# Autodesk Inventor assembly: my1020_motor
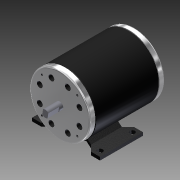
[picture p0: Inventor's stored thumbnail of the model, 180x180]
Saved by Autodesk Inventor 2012 (Build 160160000, 160)
## iProperties
Created: 2012-01-29
Part Number: my1020_motor
Document SubType Name: Assembly
Designer: Antonella Wilby
Author: Antonella Wilby
## Documents named in this file (4)
- E:\GCC Robotics 2012 - Mechanical\Robot 2.0\Drive Train\MY1020 Motor\my1020_motor.iam
- E:\GCC Robotics 2012 - Mechanical\Robot 2.0\Drive Train\MY1020 Motor\my1020_motor.ipt
- E:\GCC Robotics 2012 - Mechanical\Robot 2.0\Drive Train\MY1020 Motor\shaft.ipt
- E:\GCC Robotics 2012 - Mechanical\Robot 2.0\Drive Train\MY1020 Motor\mount plate.ipt
## Components (3 placed, 3 different names)
1. my1020_motor:1 — Mate:1, Mate:2, Mate:4, Mate:5, Flush:1
2. shaft:1 — Mate:1, Mate:2
3. mount plate:1 — Mate:4, Mate:5, Flush:1
## Relationships (5: Mate 4, Flush 1)
- Mate:1: my1020_motor:1 ↔ shaft:1
- Mate:2: my1020_motor:1 ↔ shaft:1
- Mate:4: my1020_motor:1 ↔ mount plate:1
- Mate:5: my1020_motor:1 ↔ mount plate:1
- Flush:1 (-22.225 mm): my1020_motor:1 ↔ mount plate:1
